# Autodesk Inventor assembly: Facade13
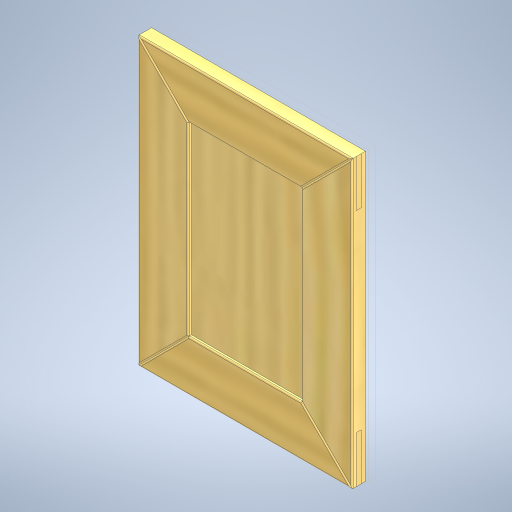
[picture p0: Inventor's stored thumbnail of the model, 512x512]
Saved by Autodesk Inventor 2024 (Build 280153000, 153)
## iProperties
RuleStatus: InUse
Created: 2019-10-01
Part Number: Facade13
Document SubType Name: Assembly
Designer: RokasM
Author: RokasM
## Documents named in this file (7)
- C:\W4INV 2024 Design\iBOX LIBRARY\Facades\Solid Wood Facade 13\Facade13.iam
- C:\W4INV 2024 Design\iBOX LIBRARY\Facades\Solid Wood Facade 13\box.ipt
- C:\W4INV 2024 Design\iBOX LIBRARY\Facades\Solid Wood Facade 13\left_profile.ipt
- C:\W4INV 2024 Design\iBOX LIBRARY\Facades\Solid Wood Facade 13\right_profile.ipt
- C:\W4INV 2024 Design\iBOX LIBRARY\Facades\Solid Wood Facade 13\top_profile.ipt
- C:\W4INV 2024 Design\iBOX LIBRARY\Facades\Solid Wood Facade 13\panel.ipt
- C:\W4INV 2024 Design\iBOX LIBRARY\Facades\Solid Wood Facade 13\Facade13.ipt
## Components (7 placed, 6 different names)
1. @Facade13
2. box:1
3. left_profile:1 — Mate:1
4. right_profile:1 — Mate:2, Flush:1
5. top_profile:1
6. panel:1
7. top_profile:2 — Mate:1, Mate:2, Flush:1
## Relationships (3: Mate 2, Flush 1)
- Mate:1: left_profile:1 ↔ top_profile:2
- Mate:2: right_profile:1 ↔ top_profile:2
- Flush:1: right_profile:1 ↔ top_profile:2
## Named parameters: offset_top = 0 mm, offset_right = 0 mm, offset_bottom = 0 mm, offset_left = 0 mm, offset_facade = 2 mm, tolerance_top = 1.5 mm, tolerance_right = 1.5 mm, tolerance_bottom = 1.5 mm, tolerance_left = 1.5 mm
